# Autodesk Inventor assembly: WithAdapter4Inch60A
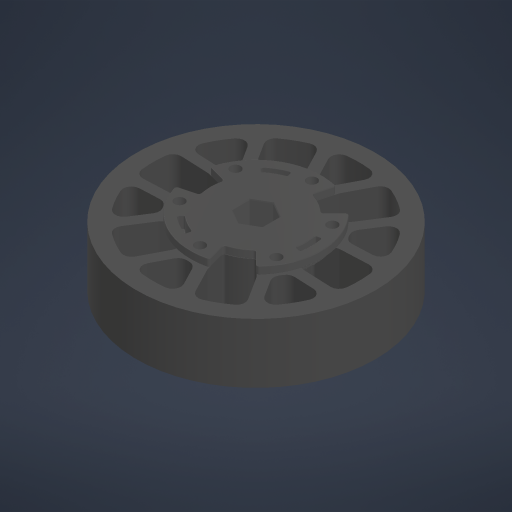
[picture p0: Inventor's stored thumbnail of the model, 512x512]
Saved by Autodesk Inventor 2023 (Build 270158000, 158)
## iProperties
Created: 2022-09-22
Part Number: WithAdapter4Inch60A
Document SubType Name: Assembly
Designer: alex
Author: alex
## Documents named in this file (4)
- C:\Users\alex\Documents\GitHub\4067X_spin_up_cad\WithAdapter4Inch60A.iam
- C:\Users\alex\Documents\GitHub\4067X_spin_up_cad\Library\Motion\Wheels\Flex Wheels\4.000 Flex Wheel\4.000 60A 1.000.ipt
- C:\Users\alex\Documents\GitHub\4067X_spin_up_cad\Library\Motion\Wheels\Flex Wheels\4.000 Flex Wheel.ipt
- C:\Users\alex\Documents\GitHub\4067X_spin_up_cad\Library\Motion\Wheels\Flex Wheels\VersaHub.ipt
## Components (3 placed, 2 different names)
1. 4.000 60A 1.000:1 — Mate:1, Mate:2, Mate:3, Mate:4, Mate:5, Mate:6
2. VersaHub:1 — Mate:1, Mate:2, Mate:3
3. VersaHub:2 — Mate:4, Mate:5, Mate:6
## Relationships (6: Mate 6)
- Mate:1: 4.000 60A 1.000:1 ↔ VersaHub:1
- Mate:2: 4.000 60A 1.000:1 ↔ VersaHub:1
- Mate:3: 4.000 60A 1.000:1 ↔ VersaHub:1
- Mate:4: 4.000 60A 1.000:1 ↔ VersaHub:2
- Mate:5: 4.000 60A 1.000:1 ↔ VersaHub:2
- Mate:6: 4.000 60A 1.000:1 ↔ VersaHub:2
